# Autodesk Inventor assembly: Assembly1
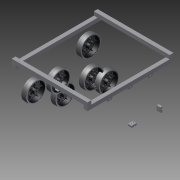
[picture p0: Inventor's stored thumbnail of the model, 180x180]
Saved by Autodesk Inventor 2015 (Build 190159000, 159)
## iProperties
Created: 2014-10-03
Part Number: Assembly1
Document SubType Name: Assembly
Designer: jesse
Author: jesse
## Documents named in this file (5)
- C:\Users\jesse\Desktop\robot\Assembly1.iam
- C:\Users\jesse\Desktop\robot\y base piece.ipt
- C:\Users\jesse\Desktop\robot\x base piece.ipt
- C:\Users\jesse\Desktop\2012_FTC_KOP\Imported Components\am-2648_4inWheel8mmHub\am-2648_4inWheel8mmHub.iam
- C:\Users\jesse\Desktop\robot\axle holder.ipt
## Components (16 placed, 4 different names)
1. y base piece:1 — Flush:1, Mate:1, Flush:2, Mate:4, Flush:7, Mate:5, Flush:8, Mate:6, Flush:10
2. x base piece:1 — Flush:1, Mate:1, Flush:2, Flush:3, Mate:2, Flush:4
3. y base piece:2 — Flush:3, Mate:2, Flush:4, Flush:5, Flush:6, Mate:3
4. x base piece:2 — Flush:5, Flush:6, Mate:3, Flush:9
5. am-2648_4inWheel8mmHub:1 [sub-assembly]
6. am-2648_4inWheel8mmHub:2 [sub-assembly]
7. am-2648_4inWheel8mmHub:3 [sub-assembly]
8. am-2648_4inWheel8mmHub:4 [sub-assembly]
9. am-2648_4inWheel8mmHub:5 [sub-assembly]
10. am-2648_4inWheel8mmHub:6 [sub-assembly]
11. axle holder:1 — Mate:4, Flush:7
12. axle holder:2 — Mate:5, Flush:8
13. axle holder:3
14. axle holder:4
15. axle holder:5 — Mate:6, Flush:10
16. axle holder:6 — Flush:9
## Relationships (16: Flush 10, Mate 6)
- Flush:1: y base piece:1 ↔ x base piece:1
- Mate:1: y base piece:1 ↔ x base piece:1
- Flush:2: y base piece:1 ↔ x base piece:1
- Flush:3: x base piece:1 ↔ y base piece:2
- Mate:2: x base piece:1 ↔ y base piece:2
- Flush:4: x base piece:1 ↔ y base piece:2
- Flush:5: y base piece:2 ↔ x base piece:2
- Flush:6: y base piece:2 ↔ x base piece:2
- Mate:3: y base piece:2 ↔ x base piece:2
- Mate:4: y base piece:1 ↔ axle holder:1
- Flush:7: y base piece:1 ↔ axle holder:1
- Mate:5: y base piece:1 ↔ axle holder:2
- Flush:8: y base piece:1 ↔ axle holder:2
- Flush:9: x base piece:2 ↔ axle holder:6
- Mate:6: y base piece:1 ↔ axle holder:5
- Flush:10: y base piece:1 ↔ axle holder:5
